# Autodesk Inventor assembly: 轮腿
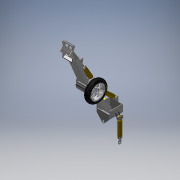
[picture p0: Inventor's stored thumbnail of the model, 180x180]
Saved by Autodesk Inventor 2019 (Build 230136000, 136)
## iProperties
Created: 2018-12-12
Part Number: 轮腿
Document SubType Name: Assembly
Designer: Administrator
Author: Administrator
## Documents named in this file (16)
- C:\Users\Administrator\Desktop\机械产品数字化设计大赛\轮腿\左轮腿.iam
- C:\Users\Administrator\Desktop\机械产品数字化设计大赛\轮腿\底座.ipt
- C:\Users\Administrator\Desktop\机械产品数字化设计大赛\轮腿\销钉400_60 .ipt
- C:\Users\Administrator\Desktop\机械产品数字化设计大赛\轮腿\液压杆体.ipt
- C:\Users\Administrator\Desktop\机械产品数字化设计大赛\轮腿\液压杆.ipt
- C:\Users\Administrator\Desktop\机械产品数字化设计大赛\轮腿\销钉340_54.ipt
- C:\Users\Administrator\Desktop\机械产品数字化设计大赛\轮腿\销钉120_60.ipt
- C:\Users\Administrator\Desktop\机械产品数字化设计大赛\轮腿\二级外壳.ipt
- C:\Users\Administrator\Desktop\机械产品数字化设计大赛\轮腿\销钉340_50.ipt
- C:\Users\Administrator\Desktop\机械产品数字化设计大赛\轮腿\末端爪.ipt
- C:\Users\Administrator\Desktop\机械产品数字化设计大赛\轮腿\末端销钉120_40.ipt
- C:\Users\Administrator\Desktop\机械产品数字化设计大赛\轮腿\销钉340_60.ipt
- C:\Users\Administrator\Desktop\机械产品数字化设计大赛\轮腿\销钉280_54.ipt
- C:\Users\Administrator\Desktop\机械产品数字化设计大赛\轮腿\轮子\HP2 Raceparts Complette Tyre.iam
- C:\Users\Administrator\Desktop\机械产品数字化设计大赛\轮腿\一级外壳右.ipt
- C:\Users\Administrator\Desktop\机械产品数字化设计大赛\轮腿\液压杆盖.ipt
## Components (22 placed, 15 different names)
1. 底座:1 — 配合:3, 配合:4, 配合:12, 配合:13, 配合:21, 配合:22, 配合:39, 表面齐平:1, 配合:49, 配合:52, 配合:53
2. 销钉400_60 :1 — 配合:38, 配合:39, 配合:49
3. 液压杆体:1 — 配合:3, 配合:4, 配合:7, 插入:2, 配合:50
4. 液压杆:1 — 配合:7, 配合:11, 配合:50
5. 销钉340_54:1 — 配合:11, 配合:40, 配合:45
6. 销钉120_60:1 — 配合:12, 配合:13
7. 二级外壳:1 — 配合:26, 配合:27, 配合:28, 配合:30, 配合:31, 配合:32, 配合:33, 配合:36, 配合:46, 角度:2
8. 销钉340_50:1 — 配合:26, 配合:47
9. 末端爪:1 — 配合:30, 配合:31, 角度:2
10. 末端销钉120_40:1 — 配合:32, 配合:33
11. 液压杆体:2 — 配合:21, 配合:22, 配合:23, 插入:1
12. 液压杆:2 — 配合:23
13. 液压杆体:3 — 配合:29, 配合:43, 配合:44, 插入:3, 配合:51
14. 液压杆:3 — 配合:27, 配合:28, 配合:29, 配合:51
15. 销钉340_60:1 — 配合:41, 配合:42, 配合:43
16. 销钉280_54:1 — 配合:36
17. HP2 Raceparts Complette Tyre:1 [sub-assembly] — 配合:48, 角度:1
18. 一级外壳右:1 — 配合:38, 表面齐平:1, 配合:40, 配合:41, 配合:42, 配合:44, 配合:45, 配合:46, 配合:47, 配合:48, 角度:1
19. 液压杆盖:1 — 插入:1
20. 液压杆盖:2 — 插入:3
21. 液压杆盖:3 — 插入:2
22. 销钉120_60:2 — 配合:52, 配合:53
## Relationships (40: Mate 34, Insert 3, Angle 2, Flush 1)
- 配合:3 [Mate]: 底座:1 ↔ 液压杆体:1
- 配合:4 [Mate]: 底座:1 ↔ 液压杆体:1
- 配合:7 [Mate]: 液压杆体:1 ↔ 液压杆:1
- 配合:11 [Mate]: 液压杆:1 ↔ 销钉340_54:1
- 配合:12 [Mate]: 底座:1 ↔ 销钉120_60:1
- 配合:13 [Mate]: 底座:1 ↔ 销钉120_60:1
- 配合:21 [Mate]: 底座:1 ↔ 液压杆体:2
- 配合:22 [Mate]: 底座:1 ↔ 液压杆体:2
- 配合:23 [Mate]: 液压杆体:2 ↔ 液压杆:2
- 配合:26 [Mate]: 二级外壳:1 ↔ 销钉340_50:1
- 配合:27 [Mate]: 二级外壳:1 ↔ 液压杆:3
- 配合:28 [Mate]: 二级外壳:1 ↔ 液压杆:3
- 配合:29 [Mate]: 液压杆体:3 ↔ 液压杆:3
- 配合:30 [Mate]: 二级外壳:1 ↔ 末端爪:1
- 配合:31 [Mate]: 二级外壳:1 ↔ 末端爪:1
- 配合:32 [Mate]: 二级外壳:1 ↔ 末端销钉120_40:1
- 配合:33 [Mate]: 二级外壳:1 ↔ 末端销钉120_40:1
- 配合:36 [Mate]: 二级外壳:1 ↔ 销钉280_54:1
- 配合:38 [Mate]: 销钉400_60 :1 ↔ 一级外壳右:1
- 配合:39 [Mate]: 底座:1 ↔ 销钉400_60 :1
- 表面齐平:1 [Flush] (30 mm): 底座:1 ↔ 一级外壳右:1
- 配合:40 [Mate]: 销钉340_54:1 ↔ 一级外壳右:1
- 配合:41 [Mate]: 销钉340_60:1 ↔ 一级外壳右:1
- 配合:42 [Mate]: 销钉340_60:1 ↔ 一级外壳右:1
- 配合:43 [Mate]: 液压杆体:3 ↔ 销钉340_60:1
- 配合:44 [Mate]: 液压杆体:3 ↔ 一级外壳右:1
- 配合:45 [Mate]: 销钉340_54:1 ↔ 一级外壳右:1
- 配合:46 [Mate]: 二级外壳:1 ↔ 一级外壳右:1
- 配合:47 [Mate]: 销钉340_50:1 ↔ 一级外壳右:1
- 配合:48 [Mate]: HP2 Raceparts Complette Tyre:1 ↔ 一级外壳右:1
- 配合:49 [Mate]: 底座:1 ↔ 销钉400_60 :1
- 角度:1 [Angle] (196 deg): HP2 Raceparts Complette Tyre:1 ↔ 一级外壳右:1
- 插入:1 [Insert]: 液压杆体:2 ↔ 液压杆盖:1
- 插入:2 [Insert]: 液压杆体:1 ↔ 液压杆盖:3
- 插入:3 [Insert]: 液压杆体:3 ↔ 液压杆盖:2
- 配合:50 [Mate]: 液压杆体:1 ↔ 液压杆:1
- 配合:51 [Mate]: 液压杆体:3 ↔ 液压杆:3
- 角度:2 [Angle] (0 deg): 二级外壳:1 ↔ 末端爪:1
- 配合:52 [Mate]: 底座:1 ↔ 销钉120_60:2
- 配合:53 [Mate]: 底座:1 ↔ 销钉120_60:2
